# Autodesk Inventor assembly: 8mm Bearing with Hex Insert_MIR
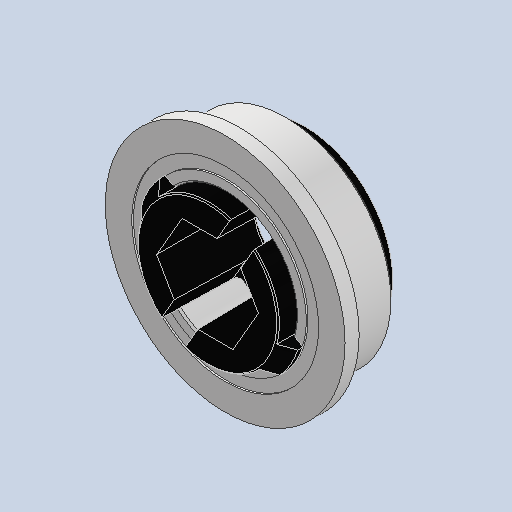
[picture p0: Inventor's stored thumbnail of the model, 512x512]
Saved by Autodesk Inventor 2022 (Build 260153000, 153)
## iProperties
Created: 2020-10-02
Part Number: 8mm Bearing with Hex Insert_MIR
Document SubType Name: Assembly
Designer: matt
Author: matt
## Documents named in this file (3)
- C:\Users\matt\Documents\Inventor\FTC\2022-23 FTC\FTC Robot Parts\Structural\8mm Bearing with Hex Insert_MIR.iam
- C:\Users\matt\Documents\Inventor\FTC\2022-23 FTC\8mm Bearing REV-49-1559_MIR.ipt
- C:\Users\matt\Documents\Inventor\FTC\2022-23 FTC\5mm Hex Bearing Insert_MIR.ipt
## Components (2 placed, 2 different names)
1. 8mm Bearing REV-49-1559_MIR:1 — Mate:2, Mate:1
2. 5mm Hex Bearing Insert_MIR:1 — Mate:2, Mate:1
## Relationships (2: Mate 2)
- Mate:2: 8mm Bearing REV-49-1559_MIR:1 ↔ 5mm Hex Bearing Insert_MIR:1
- Mate:1: 8mm Bearing REV-49-1559_MIR:1 ↔ 5mm Hex Bearing Insert_MIR:1
